# Autodesk Inventor assembly: WithoutFrame
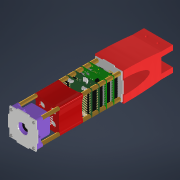
[picture p0: Inventor's stored thumbnail of the model, 180x180]
Saved by Autodesk Inventor 2022 (Build 260153000, 153)
## iProperties
Created: 2022-07-14
Part Number: WithoutFrame
Document SubType Name: Assembly
Designer: ForseFire
Author: ForseFire
## Documents named in this file (4)
- C:\Users\ForseFire\Desktop\WithoutFrame.iam
- C:\Users\ForseFire\Desktop\CameraReady.iam
- C:\Users\ForseFire\Desktop\WithoutCamera.iam
- C:\Users\ForseFire\Documents\Inventor\Content Center Files\R2022\en-US\CNS 9671\CNS 9671 - M2,6 x 20.ipt
## Components (6 placed, 3 different names)
1. WithoutCamera:1 [sub-assembly] — Mate:1, Mate:2
2. CameraReady:1 [sub-assembly] — Mate:1, Mate:2, Mate:3, Mate:4, Mate:5, Mate:6, Mate:7, Mate:8, Mate:9, Mate:10
3. CNS 9671 M2,6 x 20:1 — Mate:5, Mate:10
4. CNS 9671 M2,6 x 20:2 — Mate:4, Mate:8
5. CNS 9671 M2,6 x 20:3 — Mate:3, Mate:7
6. CNS 9671 M2,6 x 20:4 — Mate:6, Mate:9
## Relationships (10: Mate 10)
- Mate:1: WithoutCamera:1 ↔ CameraReady:1
- Mate:2: WithoutCamera:1 ↔ CameraReady:1
- Mate:3: CameraReady:1 ↔ CNS 9671 M2,6 x 20:3
- Mate:4: CameraReady:1 ↔ CNS 9671 M2,6 x 20:2
- Mate:5: CameraReady:1 ↔ CNS 9671 M2,6 x 20:1
- Mate:6: CameraReady:1 ↔ CNS 9671 M2,6 x 20:4
- Mate:7: CameraReady:1 ↔ CNS 9671 M2,6 x 20:3
- Mate:8: CameraReady:1 ↔ CNS 9671 M2,6 x 20:2
- Mate:9: CameraReady:1 ↔ CNS 9671 M2,6 x 20:4
- Mate:10: CameraReady:1 ↔ CNS 9671 M2,6 x 20:1
